# Autodesk Inventor assembly: Fanduct
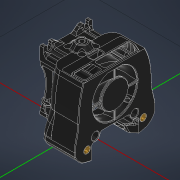
[picture p0: Inventor's stored thumbnail of the model, 180x180]
Saved by Autodesk Inventor 2022.2 (Build 262287010, 287A)
## iProperties
Created: 2022-03-16
Part Number: Fanduct
Document SubType Name: Assembly
Designer: sleib
Author: sleib
## Documents named in this file (4)
- C:\Users\sleib\Projekte\Voron-2\CAD\Inventor\Afterburner\Fanduct.iam
- C:\Users\sleib\Projekte\Voron-2\CAD\Inventor\Afterburner\Hotend Back.ipt
- C:\Users\sleib\Projekte\Voron-2\CAD\Inventor\Afterburner\Hotend Fanduct.ipt
- C:\Users\sleib\Projekte\Voron-2\CAD\Inventor\M3 Threaded Insert.ipt
## Components (4 placed, 3 different names)
1. Hotend Back:1 — Fluchtend:1, Passend:1, Passend:2, Passend:3, Fluchtend:2
2. Hotend Fanduct:1 — Fluchtend:1, Passend:1, Passend:2, Passend:3, Fluchtend:2, Passend:4, Passend:5, Fluchtend:3, Fluchtend:4
3. M3 Threaded Insert:1 — Passend:4, Fluchtend:4
4. M3 Threaded Insert:2 — Passend:5, Fluchtend:3
## Relationships (9: Mate 5, Flush 4)
- Fluchtend:1 [Flush]: Hotend Back:1 ↔ Hotend Fanduct:1
- Passend:1 [Mate]: Hotend Back:1 ↔ Hotend Fanduct:1
- Passend:2 [Mate]: Hotend Back:1 ↔ Hotend Fanduct:1
- Passend:3 [Mate]: Hotend Back:1 ↔ Hotend Fanduct:1
- Fluchtend:2 [Flush]: Hotend Back:1 ↔ Hotend Fanduct:1
- Passend:4 [Mate]: Hotend Fanduct:1 ↔ M3 Threaded Insert:1
- Passend:5 [Mate]: Hotend Fanduct:1 ↔ M3 Threaded Insert:2
- Fluchtend:3 [Flush]: Hotend Fanduct:1 ↔ M3 Threaded Insert:2
- Fluchtend:4 [Flush]: Hotend Fanduct:1 ↔ M3 Threaded Insert:1
